# Autodesk Inventor assembly: IMS-00-100
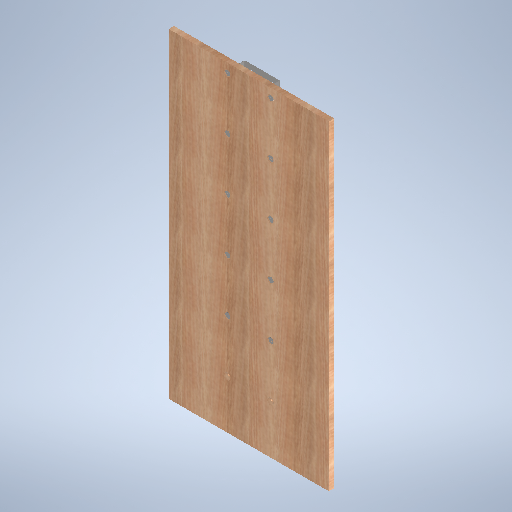
[picture p0: Inventor's stored thumbnail of the model, 512x512]
Saved by Autodesk Inventor 2025.2 (Build 292293000, 293)
## iProperties
Created: 2020-10-09
Part Number: IMS-00-100
Document SubType Name: Assembly
Designer: mahra
Author: mahra
## Documents named in this file (6)
- C:\Users\Caspe\Documents\Semester 8\Project\Anomaly_Detection\Mechanical_Project\Inventor_project\IMS-00-100.iam
- C:\Users\Caspe\Documents\Semester 8\Project\Anomaly_Detection\Mechanical_Project\Inventor_project\IMS-10-000.iam
- C:\Users\Caspe\Documents\Semester 8\Project\Anomaly_Detection\Mechanical_Project\Inventor_project\IMS-00-003.ipt
- C:\Users\Caspe\Documents\Inventor\Content Center Files\R2025\en-US\DIN 7991(2)\DIN 7991 - M10x30.ipt
- C:\Users\Caspe\Documents\Inventor\Content Center Files\R2025\en-US\DIN 1587\DIN 1587 - M10 x 1,5.ipt
- C:\Users\Caspe\Documents\Inventor\Content Center Files\R2025\en-US\DIN 125-1  A\DIN 125 - A 10,5.ipt
## Components (32 placed, 5 different names)
1. IMS-10-000:1 [sub-assembly] — Mate:20, Flush:1
2. IMS-00-003:1 — Mate:20, Flush:1, Mate:22, Flush:2
3. DIN 1587 M10 - SW16:11
4. DIN 125-1 A A 10,5:11
5. DIN 1587 M10 - SW16:16 — Insert:5
6. DIN 125-1 A A 10,5:16 — Insert:5
7. DIN 7991 M10x30:11
8. DIN 7991 M10x30:16 — Mate:22, Flush:2
9. DIN 1587 M10 - SW16:12
10. DIN 125-1 A A 10,5:12
11. DIN 1587 M10 - SW16:17
12. DIN 125-1 A A 10,5:17
13. DIN 7991 M10x30:12
14. DIN 7991 M10x30:17
15. DIN 1587 M10 - SW16:13
16. DIN 125-1 A A 10,5:13
17. DIN 1587 M10 - SW16:18
18. DIN 125-1 A A 10,5:18
19. DIN 7991 M10x30:13
20. DIN 7991 M10x30:18
21. DIN 1587 M10 - SW16:14
22. DIN 125-1 A A 10,5:14
23. DIN 1587 M10 - SW16:19
24. DIN 125-1 A A 10,5:19
25. DIN 7991 M10x30:14
26. DIN 7991 M10x30:19
27. DIN 1587 M10 - SW16:15
28. DIN 125-1 A A 10,5:15
29. DIN 1587 M10 - SW16:20
30. DIN 125-1 A A 10,5:20
31. DIN 7991 M10x30:15
32. DIN 7991 M10x30:20
## Component patterns: (5 elements, first: DIN 1587 M10 - SW16:11 + DIN 125-1 A A 10,5:11 + DIN 1587 M10 - SW16:16 + DIN 125-1 A A 10,5:16 + DIN 7991 M10x30:11 + DIN 7991 M10x30:16)
## Relationships (7: Insert 3, Mate 2, Flush 2)
- Mate:20: IMS-10-000:1 ↔ IMS-00-003:1
- Flush:1 (10 mm): IMS-10-000:1 ↔ IMS-00-003:1
- Mate:22: IMS-00-003:1 ↔ DIN 7991 M10x30:16
- Flush:2 (1.5 mm): IMS-00-003:1 ↔ DIN 7991 M10x30:16
- [Insert]: IMS-10-000:1 ↔ DIN 125-1 A A 10,5:11
- [Insert]: DIN 1587 M10 - SW16:11 ↔ DIN 125-1 A A 10,5:11
- Insert:5: DIN 1587 M10 - SW16:16 ↔ DIN 125-1 A A 10,5:16
